# Autodesk Inventor assembly: Pancake_Top Board Assy_3 Lanes
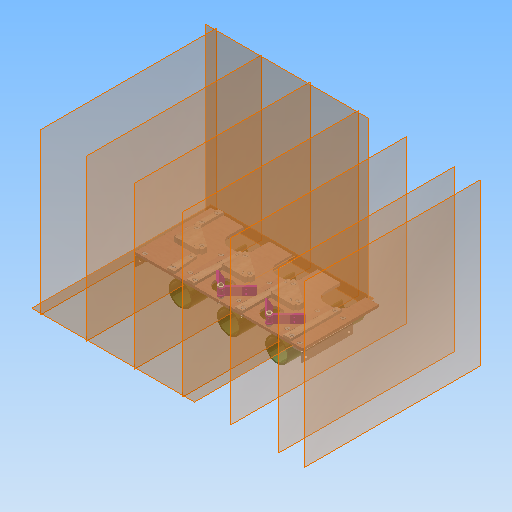
[picture p0: Inventor's stored thumbnail of the model, 512x512]
Saved by Autodesk Inventor 2018.1 (Build 221171000, 171)
## iProperties
Created: 2019-02-21
Part Number: Pancake_Top Board Assy_3 Lanes
Document SubType Name: Assembly
Designer: James
Author: James
## Documents named in this file (18)
- C:\Users\admin\Desktop\Ball-Machine\Pancake Sort\Pancake - 3 Lanes\Pancake_Top Board Assy_3 Lanes.iam
- C:\Users\admin\Desktop\Ball-Machine\Pancake Sort\Pancake_Angle Bracket 2.ipt
- C:\Users\admin\Desktop\Ball-Machine\Prototype CAD\Selection Sort - 40mm\Nyloc Nut - M4.ipt
- C:\Users\admin\Desktop\Ball-Machine\Prototype CAD\Selection Sort - 40mm\Socket Csk Screw - (A2) - M4 x  12.ipt
- C:\Users\admin\Desktop\Ball-Machine\Pancake Sort\Pancake_Side Piece.ipt
- C:\Users\admin\Desktop\Ball-Machine\Prototype CAD\Selection Sort - 40mm\Socket Csk Screw - (A2) - M4 x  16.ipt
- C:\Users\admin\Desktop\Ball-Machine\Pancake Sort\Pancake_Side Piece Short.ipt
- C:\Users\admin\Desktop\Ball-Machine\Pancake Sort\Pancake_Lower Pipe.ipt
- C:\Users\admin\Desktop\Ball-Machine\Pancake Sort\Pancake_Side Piece Short 2.ipt
- C:\Users\admin\Desktop\Ball-Machine\Pancake Sort\Socket Csk Screw - (A2) - M4 x  20.ipt
- C:\Users\admin\Desktop\Ball-Machine\Pancake Sort\Pancake_Side Piece Short 3.ipt
- C:\Users\admin\Desktop\Ball-Machine\Pancake Sort\Pancake_Switch Lever.ipt
- C:\Users\admin\Desktop\Ball-Machine\Pancake Sort\Pancake_Lever Mount Piece.ipt
- C:\Users\admin\Desktop\Ball-Machine\Selection Sort\Selection_Washer.ipt
- C:\Users\admin\Desktop\Ball-Machine\Pancake Sort\Socket Csk Screw - (A2) - M3 x  10.ipt
- C:\Users\admin\Desktop\Ball-Machine\Prototype CAD\Selection Sort - 40mm\Socket Cap Screw - Standard - (A2) - M3 x 8.ipt
- C:\Users\admin\Desktop\Ball-Machine\Pancake Sort\Pancake_Eye Screw.ipt
- C:\Users\admin\Desktop\Ball-Machine\Pancake Sort\Pancake - 3 Lanes\Pancake_Top Board_3 Lanes.ipt
## Components (80 placed, 17 different names)
1. Pancake_Top Board_3 Lanes:1 — Flush:1, Flush:2, Flush:3, Mate:1, Mate:2, Mate:3, Flush:4, Mate:4, Mate:5, Mate:6, Flush:5, Mate:7, Mate:8, Tangent:1, Tangent:2, Mate:13, Mate:14, Tangent:3, Tangent:4, Mate:19, Mate:20, Mate:21, Flush:6, Mate:24, Mate:25, Mate:28, Mate:29, Mate:30, Mate:35, Mate:36, Tangent:9, Mate:37, Mate:38, Angle:1, Mate:41, Mate:42, Tangent:10, Tangent:11, Mate:43, Mate:44, Mate:45, Mate:46, Mate:47, Mate:48, Mate:49, Mate:50, Mate:53, Mate:54, Mate:55, Mate:60, Mate:61, Mate:63, Mate:76, Mate:77, Mate:81, Tangent:19, Mate:84, Mate:85, Mate:86, Mate:87
2. Pancake_Angle Bracket 2:1 — Mate:1, Mate:2, Mate:3, Flush:4, Mate:9, Mate:10
3. Pancake_Angle Bracket 2:2 — Mate:4, Mate:5, Mate:6, Flush:5, Mate:15, Mate:16
4. Pancake_Side Piece Short 2:1 — Mate:44, Mate:45, Mate:46, Tangent:12, Tangent:13
5. Nyloc Nut - M4:35 — Mate:49, Mate:52
6. Socket Csk Screw - (A2) - M4 x  16:11 — Mate:47, Tangent:12, Mate:51
7. Nyloc Nut - M4:36 — Mate:50, Mate:51
8. Socket Csk Screw - (A2) - M4 x  16:12 — Mate:48, Tangent:13, Mate:52
9. Pancake_Side Piece Short 3:1 — Mate:53, Mate:54, Mate:55, Mate:58, Mate:59, Tangent:14, Tangent:15
10. Socket Csk Screw - (A2) - M4 x  16:13 — Mate:58, Tangent:14
11. Nyloc Nut - M4:37 — Mate:61
12. Socket Csk Screw - (A2) - M4 x  16:14 — Mate:59, Tangent:15
13. Nyloc Nut - M4:38 — Mate:60
14. Nyloc Nut - M4:1 — Mate:9, Mate:12
15. Nyloc Nut - M4:2 — Mate:10, Mate:11
16. Nyloc Nut - M4:3 — Mate:16, Mate:18
17. Nyloc Nut - M4:4 — Mate:15, Mate:17
18. Socket Csk Screw - (A2) - M4 x  12:1 — Mate:7, Tangent:1, Mate:11
19. Socket Csk Screw - (A2) - M4 x  12:2 — Mate:8, Tangent:2, Mate:12
20. Socket Csk Screw - (A2) - M4 x  12:3 — Mate:14, Tangent:3, Mate:17
21. Socket Csk Screw - (A2) - M4 x  12:4 — Mate:13, Tangent:4, Mate:18
22. Socket Csk Screw - (A2) - M4 x  16:2 — Mate:23, Tangent:5, Mate:27
23. Nyloc Nut - M4:6 — Mate:25, Mate:27
24. Socket Csk Screw - (A2) - M4 x  16:1 — Mate:22, Tangent:6, Mate:26
25. Nyloc Nut - M4:5 — Mate:24, Mate:26
26. Pancake_Side Piece:1 — Mate:19, Mate:20, Mate:21, Flush:6, Mate:22, Mate:23, Tangent:5, Tangent:6
27. Socket Csk Screw - (A2) - M4 x  16:3
28. Nyloc Nut - M4:7
29. Socket Csk Screw - (A2) - M4 x  16:4
30. Nyloc Nut - M4:8
31. Pancake_Side Piece:2 — Tangent:16
32. Socket Csk Screw - (A2) - M4 x  16:5
33. Nyloc Nut - M4:9
34. Socket Csk Screw - (A2) - M4 x  16:6
35. Nyloc Nut - M4:10
36. Pancake_Side Piece:3
37. Pancake_Side Piece Short:1 — Mate:28, Mate:29, Mate:30, Mate:33, Mate:34, Tangent:7, Tangent:8
38. Nyloc Nut - M4:15 — Mate:36
39. Socket Csk Screw - (A2) - M4 x  20:1 — Mate:34, Tangent:7
40. Nyloc Nut - M4:16 — Mate:35
41. Socket Csk Screw - (A2) - M4 x  20:6 — Mate:33, Tangent:8
42. Pancake_Side Piece Short:2 — Tangent:18, Mate:88, Mate:89
43. Nyloc Nut - M4:17
44. Socket Csk Screw - (A2) - M4 x  20:2
45. Nyloc Nut - M4:18
46. Socket Csk Screw - (A2) - M4 x  20:7
47. Pancake_Side Piece Short:3
48. Nyloc Nut - M4:19
49. Socket Csk Screw - (A2) - M4 x  20:3
50. Nyloc Nut - M4:20
51. Socket Csk Screw - (A2) - M4 x  20:8
52. Socket Csk Screw - (A2) - M4 x  12:6 — Mate:42, Tangent:11
53. Nyloc Nut - M4:26 — Mate:43, Flush:8
54. Socket Csk Screw - (A2) - M4 x  12:5 — Mate:41, Tangent:10
55. Nyloc Nut - M4:25 — Flush:8
56. Pancake_Lower Pipe:1 — Tangent:9, Mate:37, Mate:38, Angle:1
57. Socket Csk Screw - (A2) - M4 x  12:7
58. Nyloc Nut - M4:27
59. Socket Csk Screw - (A2) - M4 x  12:8
60. Nyloc Nut - M4:28
61. Pancake_Lower Pipe:2
62. Socket Csk Screw - (A2) - M4 x  12:9
63. Nyloc Nut - M4:29
64. Socket Csk Screw - (A2) - M4 x  12:10
65. Nyloc Nut - M4:30
66. Pancake_Lower Pipe:3
67. Socket Cap Screw - Standard - (A2) - M3 x 8:1 — Mate:82, Mate:83
68. Selection_Washer:2 — Mate:78, Mate:79, Mate:82, Mate:83
69. Pancake_Switch Lever:1 — Mate:63, Tangent:16, Tangent:18, Mate:80
70. Socket Csk Screw - (A2) - M3 x  10:2 — Mate:81, Tangent:19
71. Pancake_Lever Mount Piece:2 — Mate:76, Mate:77, Mate:78, Mate:79, Mate:80
72. Pancake_Eye Screw:7 — Mate:88, Mate:89
73. Socket Cap Screw - Standard - (A2) - M3 x 8:2
74. Selection_Washer:3
75. Pancake_Switch Lever:2
76. Socket Csk Screw - (A2) - M3 x  10:3
77. Pancake_Lever Mount Piece:3
78. Pancake_Eye Screw:8
79. Pancake_Eye Screw:1 — Mate:84, Mate:85
80. Pancake_Eye Screw:2 — Mate:86, Mate:87
## Component patterns: (3 elements, first: Socket Csk Screw - (A2) - M4 x  16:2 + Nyloc Nut - M4:6 + Socket Csk Screw - (A2) - M4 x  16:1 + Nyloc Nut - M4:5 + Pancake_Side Piece:1), (3 elements, first: Pancake_Side Piece Short:1 + Nyloc Nut - M4:15 + Socket Csk Screw - (A2) - M4 x  20:1 + Nyloc Nut - M4:16 + Socket Csk Screw - (A2) - M4 x  20:6), (3 elements, first: Socket Csk Screw - (A2) - M4 x  12:6 + Nyloc Nut - M4:26 + Socket Csk Screw - (A2) - M4 x  12:5 + Nyloc Nut - M4:25 + Pancake_Lower Pipe:1), (2 elements, first: Socket Cap Screw - Standard - (A2) - M3 x 8:1 + Selection_Washer:2 + Pancake_Switch Lever:1 + Socket Csk Screw - (A2) - M3 x  10:2 + Pancake_Lever Mount Piece:2 + Pancake_Eye Screw:7), (1 elements, first: Pancake_Eye Screw:1 + Pancake_Eye Screw:2)
## Relationships (102: Mate 76, Tangent 18, Flush 7, Angle 1)
- Flush:1: Pancake_Top Board_3 Lanes:1
- Flush:2: Pancake_Top Board_3 Lanes:1
- Flush:3: Pancake_Top Board_3 Lanes:1
- Mate:1: Pancake_Top Board_3 Lanes:1 ↔ Pancake_Angle Bracket 2:1
- Mate:2: Pancake_Top Board_3 Lanes:1 ↔ Pancake_Angle Bracket 2:1
- Mate:3: Pancake_Top Board_3 Lanes:1 ↔ Pancake_Angle Bracket 2:1
- Flush:4: Pancake_Top Board_3 Lanes:1 ↔ Pancake_Angle Bracket 2:1
- Mate:4: Pancake_Top Board_3 Lanes:1 ↔ Pancake_Angle Bracket 2:2
- Mate:5: Pancake_Top Board_3 Lanes:1 ↔ Pancake_Angle Bracket 2:2
- Mate:6: Pancake_Top Board_3 Lanes:1 ↔ Pancake_Angle Bracket 2:2
- Flush:5: Pancake_Top Board_3 Lanes:1 ↔ Pancake_Angle Bracket 2:2
- Mate:7: Pancake_Top Board_3 Lanes:1 ↔ Socket Csk Screw - (A2) - M4 x  12:1
- Mate:8: Pancake_Top Board_3 Lanes:1 ↔ Socket Csk Screw - (A2) - M4 x  12:2
- Tangent:1: Pancake_Top Board_3 Lanes:1 ↔ Socket Csk Screw - (A2) - M4 x  12:1
- Tangent:2: Pancake_Top Board_3 Lanes:1 ↔ Socket Csk Screw - (A2) - M4 x  12:2
- Mate:9: Pancake_Angle Bracket 2:1 ↔ Nyloc Nut - M4:1
- Mate:10: Pancake_Angle Bracket 2:1 ↔ Nyloc Nut - M4:2
- Mate:11: Nyloc Nut - M4:2 ↔ Socket Csk Screw - (A2) - M4 x  12:1
- Mate:12: Nyloc Nut - M4:1 ↔ Socket Csk Screw - (A2) - M4 x  12:2
- Mate:13: Pancake_Top Board_3 Lanes:1 ↔ Socket Csk Screw - (A2) - M4 x  12:4
- Mate:14: Pancake_Top Board_3 Lanes:1 ↔ Socket Csk Screw - (A2) - M4 x  12:3
- Tangent:3: Pancake_Top Board_3 Lanes:1 ↔ Socket Csk Screw - (A2) - M4 x  12:3
- Tangent:4: Pancake_Top Board_3 Lanes:1 ↔ Socket Csk Screw - (A2) - M4 x  12:4
- Mate:15: Pancake_Angle Bracket 2:2 ↔ Nyloc Nut - M4:4
- Mate:16: Pancake_Angle Bracket 2:2 ↔ Nyloc Nut - M4:3
- Mate:17: Nyloc Nut - M4:4 ↔ Socket Csk Screw - (A2) - M4 x  12:3
- Mate:18: Nyloc Nut - M4:3 ↔ Socket Csk Screw - (A2) - M4 x  12:4
- Mate:19: Pancake_Top Board_3 Lanes:1 ↔ Pancake_Side Piece:1
- Mate:20: Pancake_Top Board_3 Lanes:1 ↔ Pancake_Side Piece:1
- Mate:21: Pancake_Top Board_3 Lanes:1 ↔ Pancake_Side Piece:1
- Flush:6: Pancake_Top Board_3 Lanes:1 ↔ Pancake_Side Piece:1
- Mate:22: Socket Csk Screw - (A2) - M4 x  16:1 ↔ Pancake_Side Piece:1
- Mate:23: Socket Csk Screw - (A2) - M4 x  16:2 ↔ Pancake_Side Piece:1
- Tangent:5: Socket Csk Screw - (A2) - M4 x  16:2 ↔ Pancake_Side Piece:1
- Tangent:6: Socket Csk Screw - (A2) - M4 x  16:1 ↔ Pancake_Side Piece:1
- Mate:24: Pancake_Top Board_3 Lanes:1 ↔ Nyloc Nut - M4:5
- Mate:25: Pancake_Top Board_3 Lanes:1 ↔ Nyloc Nut - M4:6
- Mate:26: Socket Csk Screw - (A2) - M4 x  16:1 ↔ Nyloc Nut - M4:5
- Mate:27: Socket Csk Screw - (A2) - M4 x  16:2 ↔ Nyloc Nut - M4:6
- Mate:28: Pancake_Top Board_3 Lanes:1 ↔ Pancake_Side Piece Short:1
- Mate:29: Pancake_Top Board_3 Lanes:1 ↔ Pancake_Side Piece Short:1
- Mate:30: Pancake_Top Board_3 Lanes:1 ↔ Pancake_Side Piece Short:1
- [Mate]: Nyloc Nut - M4:15 ↔ Socket Csk Screw - (A2) - M4 x  20:1
- [Mate]: Nyloc Nut - M4:16 ↔ Socket Csk Screw - (A2) - M4 x  20:6
- Mate:33: Pancake_Side Piece Short:1 ↔ Socket Csk Screw - (A2) - M4 x  20:6
- Mate:34: Pancake_Side Piece Short:1 ↔ Socket Csk Screw - (A2) - M4 x  20:1
- Tangent:7: Pancake_Side Piece Short:1 ↔ Socket Csk Screw - (A2) - M4 x  20:1
- Tangent:8: Pancake_Side Piece Short:1 ↔ Socket Csk Screw - (A2) - M4 x  20:6
- Mate:35: Pancake_Top Board_3 Lanes:1 ↔ Nyloc Nut - M4:16
- Mate:36: Pancake_Top Board_3 Lanes:1 ↔ Nyloc Nut - M4:15
- Tangent:9: Pancake_Top Board_3 Lanes:1 ↔ Pancake_Lower Pipe:1
- Mate:37: Pancake_Top Board_3 Lanes:1 ↔ Pancake_Lower Pipe:1
- Mate:38: Pancake_Top Board_3 Lanes:1 ↔ Pancake_Lower Pipe:1
- Angle:1 (180 deg): Pancake_Top Board_3 Lanes:1 ↔ Pancake_Lower Pipe:1
- [Mate]: Socket Csk Screw - (A2) - M4 x  12:5 ↔ Nyloc Nut - M4:25
- [Mate]: Socket Csk Screw - (A2) - M4 x  12:6 ↔ Nyloc Nut - M4:26
- Mate:41: Pancake_Top Board_3 Lanes:1 ↔ Socket Csk Screw - (A2) - M4 x  12:5
- Mate:42: Pancake_Top Board_3 Lanes:1 ↔ Socket Csk Screw - (A2) - M4 x  12:6
- Tangent:10: Pancake_Top Board_3 Lanes:1 ↔ Socket Csk Screw - (A2) - M4 x  12:5
- Tangent:11: Pancake_Top Board_3 Lanes:1 ↔ Socket Csk Screw - (A2) - M4 x  12:6
- Mate:43 (3 mm): Pancake_Top Board_3 Lanes:1 ↔ Nyloc Nut - M4:26
- Flush:8: Nyloc Nut - M4:26 ↔ Nyloc Nut - M4:25
- Mate:44: Pancake_Top Board_3 Lanes:1 ↔ Pancake_Side Piece Short 2:1
- Mate:45: Pancake_Top Board_3 Lanes:1 ↔ Pancake_Side Piece Short 2:1
- Mate:46: Pancake_Top Board_3 Lanes:1 ↔ Pancake_Side Piece Short 2:1
- Mate:47: Pancake_Top Board_3 Lanes:1 ↔ Socket Csk Screw - (A2) - M4 x  16:11
- Mate:48: Pancake_Top Board_3 Lanes:1 ↔ Socket Csk Screw - (A2) - M4 x  16:12
- Tangent:12: Pancake_Side Piece Short 2:1 ↔ Socket Csk Screw - (A2) - M4 x  16:11
- Tangent:13: Pancake_Side Piece Short 2:1 ↔ Socket Csk Screw - (A2) - M4 x  16:12
- Mate:49: Pancake_Top Board_3 Lanes:1 ↔ Nyloc Nut - M4:35
- Mate:50: Pancake_Top Board_3 Lanes:1 ↔ Nyloc Nut - M4:36
- Mate:51: Socket Csk Screw - (A2) - M4 x  16:11 ↔ Nyloc Nut - M4:36
- Mate:52: Nyloc Nut - M4:35 ↔ Socket Csk Screw - (A2) - M4 x  16:12
- Mate:53: Pancake_Top Board_3 Lanes:1 ↔ Pancake_Side Piece Short 3:1
- Mate:54: Pancake_Top Board_3 Lanes:1 ↔ Pancake_Side Piece Short 3:1
- Mate:55: Pancake_Top Board_3 Lanes:1 ↔ Pancake_Side Piece Short 3:1
- [Mate]: Socket Csk Screw - (A2) - M4 x  16:13 ↔ Nyloc Nut - M4:37
- [Mate]: Socket Csk Screw - (A2) - M4 x  16:14 ↔ Nyloc Nut - M4:38
- Mate:58: Pancake_Side Piece Short 3:1 ↔ Socket Csk Screw - (A2) - M4 x  16:13
- Mate:59: Pancake_Side Piece Short 3:1 ↔ Socket Csk Screw - (A2) - M4 x  16:14
- Tangent:14: Pancake_Side Piece Short 3:1 ↔ Socket Csk Screw - (A2) - M4 x  16:13
- Tangent:15: Pancake_Side Piece Short 3:1 ↔ Socket Csk Screw - (A2) - M4 x  16:14
- Mate:60: Pancake_Top Board_3 Lanes:1 ↔ Nyloc Nut - M4:38
- Mate:61: Pancake_Top Board_3 Lanes:1 ↔ Nyloc Nut - M4:37
- Mate:63: Pancake_Top Board_3 Lanes:1 ↔ Pancake_Switch Lever:1
- Tangent:16: Pancake_Side Piece:2 ↔ Pancake_Switch Lever:1
- Tangent:18: Pancake_Side Piece Short:2 ↔ Pancake_Switch Lever:1
- Mate:76: Pancake_Top Board_3 Lanes:1 ↔ Pancake_Lever Mount Piece:2
- Mate:77: Pancake_Top Board_3 Lanes:1 ↔ Pancake_Lever Mount Piece:2
- Mate:78: Selection_Washer:2 ↔ Pancake_Lever Mount Piece:2
- Mate:79: Selection_Washer:2 ↔ Pancake_Lever Mount Piece:2
- Mate:80: Pancake_Switch Lever:1 ↔ Pancake_Lever Mount Piece:2
- Mate:81: Pancake_Top Board_3 Lanes:1 ↔ Socket Csk Screw - (A2) - M3 x  10:2
- Tangent:19: Pancake_Top Board_3 Lanes:1 ↔ Socket Csk Screw - (A2) - M3 x  10:2
- Mate:82: Socket Cap Screw - Standard - (A2) - M3 x 8:1 ↔ Selection_Washer:2
- Mate:83: Socket Cap Screw - Standard - (A2) - M3 x 8:1 ↔ Selection_Washer:2
- Mate:84: Pancake_Top Board_3 Lanes:1 ↔ Pancake_Eye Screw:1
- Mate:85: Pancake_Top Board_3 Lanes:1 ↔ Pancake_Eye Screw:1
- Mate:86: Pancake_Top Board_3 Lanes:1 ↔ Pancake_Eye Screw:2
- Mate:87: Pancake_Top Board_3 Lanes:1 ↔ Pancake_Eye Screw:2
- Mate:88: Pancake_Side Piece Short:2 ↔ Pancake_Eye Screw:7
- Mate:89: Pancake_Side Piece Short:2 ↔ Pancake_Eye Screw:7
## Named parameters: d47_d39 = 0 mm, d48_d39 = 0 mm, d63_d18 = 0 mm, d64_d18 = 0 mm, d89_d84 = 0 mm, d90_d84 = 0 mm
